# Autodesk Inventor assembly: CCM_Unit_C
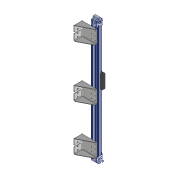
[picture p0: Inventor's stored thumbnail of the model, 180x180]
Saved by Autodesk Inventor 2020 (Build 240168000, 168)
## iProperties
Created: 2021-02-24
Part Number: CCM_Unit_C
Document SubType Name: Assembly
Designer: magnarecta
Author: magnarecta
## Documents named in this file (6)
- D:\Document\Github\Eto_Project\Hardware\Parts\CCM\CCM motion linear guide rail\CCM_UNIT\CCM_Unit_C.iam
- D:\Document\Github\Eto_Project\Hardware\Parts\CCM\CCM motion linear guide rail\CCM_UNIT\TAILSTOCK W40-00_0+0.ipt
- D:\Document\Github\Eto_Project\Hardware\Parts\CCM\CCM motion linear guide rail\CCM_UNIT\CART HK32-06W-00__1.ipt
- D:\Document\Github\Eto_Project\Hardware\Parts\CCM\CCM motion linear guide rail\CCM_UNIT\RAIL W40-06_B.ipt
- D:\Document\Github\Eto_Project\Hardware\Parts\CCM\CCM motion linear guide rail\CCM_UNIT\TAILSTOCK W40-00_0+22_1_MIR1.ipt
- D:\Document\Github\Eto_Project\Hardware\Parts\Meviy\New_Meviy\CCM_Mount_A.ipt
## Components (7 placed, 5 different names)
1. RAIL W40-06_B:1 — メイト:2, フラッシュ:3, フラッシュ:4, スライダ:1, メイト:3, フラッシュ:5, フラッシュ:6, フラッシュ:9, フラッシュ:10, メイト:6
2. TAILSTOCK W40-00_0+0:1 — メイト:2, フラッシュ:3, フラッシュ:4, メイト:5
3. CART HK32-06W-00__1:1 — スライダ:1
4. TAILSTOCK W40-00_0+22_1_MIR1:1 — メイト:3, フラッシュ:5, フラッシュ:6, メイト:4, フラッシュ:7
5. CCM_Mount_A:1 — メイト:4, フラッシュ:7, フラッシュ:8, フラッシュ:10, フラッシュ:11
6. CCM_Mount_A:2 — メイト:5, フラッシュ:8, フラッシュ:9
7. CCM_Mount_A:3 — メイト:6, フラッシュ:11
## Relationships (15: Flush 9, Mate 5, TranslationJoint 1)
- メイト:2 [Mate]: RAIL W40-06_B:1 ↔ TAILSTOCK W40-00_0+0:1
- フラッシュ:3 [Flush]: RAIL W40-06_B:1 ↔ TAILSTOCK W40-00_0+0:1
- フラッシュ:4 [Flush]: RAIL W40-06_B:1 ↔ TAILSTOCK W40-00_0+0:1
- スライダ:1 [TranslationJoint]: RAIL W40-06_B:1 ↔ CART HK32-06W-00__1:1
- メイト:3 [Mate]: RAIL W40-06_B:1 ↔ TAILSTOCK W40-00_0+22_1_MIR1:1
- フラッシュ:5 [Flush]: RAIL W40-06_B:1 ↔ TAILSTOCK W40-00_0+22_1_MIR1:1
- フラッシュ:6 [Flush]: RAIL W40-06_B:1 ↔ TAILSTOCK W40-00_0+22_1_MIR1:1
- メイト:4 [Mate]: TAILSTOCK W40-00_0+22_1_MIR1:1 ↔ CCM_Mount_A:1
- フラッシュ:7 [Flush] (-3.5 mm): TAILSTOCK W40-00_0+22_1_MIR1:1 ↔ CCM_Mount_A:1
- メイト:5 [Mate]: TAILSTOCK W40-00_0+0:1 ↔ CCM_Mount_A:2
- フラッシュ:8 [Flush]: CCM_Mount_A:1 ↔ CCM_Mount_A:2
- フラッシュ:9 [Flush]: RAIL W40-06_B:1 ↔ CCM_Mount_A:2
- フラッシュ:10 [Flush]: RAIL W40-06_B:1 ↔ CCM_Mount_A:1
- メイト:6 [Mate]: RAIL W40-06_B:1 ↔ CCM_Mount_A:3
- フラッシュ:11 [Flush]: CCM_Mount_A:1 ↔ CCM_Mount_A:3
